# Autodesk Inventor assembly: teensy_4.0
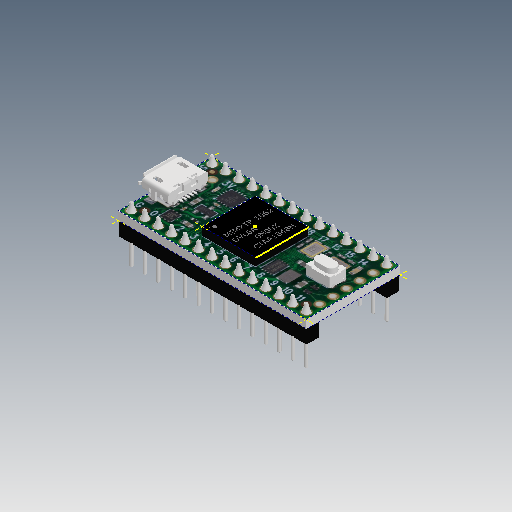
[picture p0: Inventor's stored thumbnail of the model, 512x512]
Saved by Autodesk Inventor 2020 (Build 240168000, 168)
## iProperties
Created: 2019-10-27
Part Number: teensy_4.0
Description: STEP AP203
Document SubType Name: Assembly
Designer: DELL
Sending System: SolidWorks 2019
Preprocessor: SwSTEP 2.0
Title: Teensy_4.0_Assembly.STEP
Revision Number: ANY
## Documents named in this file (7)
- F:\SoftRobot\Model\FlexipodHardware-master\mechanical_model\teensy_4.0\teensy_4.0.iam
- F:\SoftRobot\Model\FlexipodHardware-master\mechanical_model\teensy_4.0\Teensy_4.0_PCB.ipt
- F:\SoftRobot\Model\FlexipodHardware-master\mechanical_model\teensy_4.0\Micro USB-B Female 5Pin SMD.ipt
- F:\SoftRobot\Model\FlexipodHardware-master\mechanical_model\teensy_4.0\NXP iMXRT1062.ipt
- F:\SoftRobot\Model\FlexipodHardware-master\mechanical_model\teensy_4.0\SKRPACE010 v4.ipt
- F:\SoftRobot\Model\FlexipodHardware-master\mechanical_model\pins.ipt
- F:\SoftRobot\Model\FlexipodHardware-master\mechanical_model\pins_MIR1.ipt
## Components (32 placed, 6 different names)
1. Teensy_4.0_PCB_1 — Mate:1, Mate:2
2. Micro USB-B Female 5Pin SMD_2
3. NXP iMXRT1062_3
4. SKRPACE010 v4_4
5. pins_MIR1:1
6. pins_MIR1:2
7. pins_MIR1:3
8. pins_MIR1:4
9. pins_MIR1:5
10. pins_MIR1:6
11. pins_MIR1:7
12. pins_MIR1:8
13. pins_MIR1:9
14. pins_MIR1:10
15. pins_MIR1:11
16. pins_MIR1:12
17. pins_MIR1:13
18. pins_MIR1:14
19. pins:1 — Mate:1, Mate:2
20. pins:2
21. pins:3
22. pins:4
23. pins:5
24. pins:6
25. pins:7
26. pins:8
27. pins:9
28. pins:10
29. pins:11
30. pins:12
31. pins:13
32. pins:14
## Component patterns: (14 elements, first: pins:1)
## Relationships (2: Mate 2)
- Mate:1: Teensy_4.0_PCB_1 ↔ pins:1
- Mate:2: Teensy_4.0_PCB_1 ↔ pins:1
